# Autodesk Inventor assembly: standard-vslot-plate
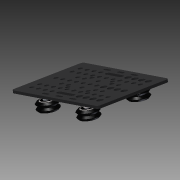
[picture p0: Inventor's stored thumbnail of the model, 180x180]
Saved by Autodesk Inventor 2015 (Build 190159000, 159)
## iProperties
Created: 2013-10-04
Part Number: standard-vslot-plate
Document SubType Name: Assembly
Designer: Michael
Author: Michael
## Documents named in this file (4)
- C:\Users\Michael\Dropbox\autocad\openbuild\standard-vslot-plate.iam
- C:\Users\Michael\Dropbox\autocad\openbuild\parts\V-Slot Solid Works\Plates\Imported Components\universal_plate\universal_plate.ipt
- C:\Users\Michael\Dropbox\autocad\openbuild\parts\standardWheel.iam
- C:\Users\Michael\Dropbox\autocad\openbuild\parts\eccentricWheel.iam
## Components (5 placed, 3 different names)
1. universal_plate:1 — Insert:1, Insert:2, Insert:3, Insert:4
2. standardWheel:1 [sub-assembly] — Insert:3
3. standardWheel:2 [sub-assembly] — Insert:4
4. eccentricWheel:1 [sub-assembly] — Insert:2
5. eccentricWheel:2 [sub-assembly] — Insert:1
## Relationships (4: Insert 4)
- Insert:1: universal_plate:1 ↔ eccentricWheel:2
- Insert:2: universal_plate:1 ↔ eccentricWheel:1
- Insert:3: universal_plate:1 ↔ standardWheel:1
- Insert:4: universal_plate:1 ↔ standardWheel:2
